# Autodesk Inventor assembly: Wheel 42T and 34T
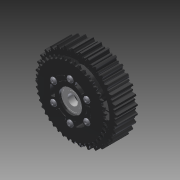
[picture p0: Inventor's stored thumbnail of the model, 180x180]
Saved by Autodesk Inventor 2013 (Build 170138000, 138)
## iProperties
Created: 2013-02-02
Part Number: Wheel 42T and 34T
Document SubType Name: Assembly
Designer: Niemitalo_Dan
Author: Niemitalo_Dan
## Documents named in this file (7)
- \\lmss\STUDENTS\Robotics\CAD Files\COTS Parts\Kit Frame - VexPro\Wheel 42T and 34T drive in a day.iam
- \\lmss\STUDENTS\Robotics\CAD Files\COTS Parts\Wheels\VexPro VersaWheel 4in.ipt
- \\lmss\STUDENTS\Robotics\CAD Files\COTS Parts\Sprockets - VexPro #25\25 Sprocket 34T Vex.ipt
- \\lmss\STUDENTS\Robotics\CAD Files\COTS Parts\Sprockets - VexPro #25\25 Sprocket 42T Vex.ipt
- \\lmss\STUDENTS\Robotics\CAD Files\COTS Parts\Fasteners\8-32 locknut.ipt
- \\lmss\STUDENTS\Robotics\CAD Files\COTS Parts\Fasteners\8-32 BHCS x2000.ipt
- \\lmss\STUDENTS\Robotics\CAD Files\COTS Parts\Bearings - VexPro\Flanged Bearing - 0.5in Round ID x 1.125in OD.ipt
## Components (17 placed, 6 different names)
1. VexPro VersaWheel 4in:1 — Mate:1, Mate:2, Mate:3, Mate:4, Mate:5, Mate:6, Mate:7, Mate:8, Mate:9, Mate:10
2. 25 Sprocket 34T Vex:1 — Mate:1, Mate:2, Mate:3, Insert:3
3. 25 Sprocket 42T Vex:1 — Mate:4, Mate:5, Mate:6, Insert:4
4. Flanged Bearing - 0.5in Round ID x 1.125in OD:1 — Mate:7, Mate:8
5. Flanged Bearing - 0.5in Round ID x 1.125in OD:2 — Mate:9, Mate:10
6. 8-32 BHCS x2000:1 — Insert:4
7. 8-32 locknut:1 — Insert:3
8. 8-32 BHCS x2000:2
9. 8-32 locknut:2
10. 8-32 BHCS x2000:3
11. 8-32 locknut:3
12. 8-32 BHCS x2000:4
13. 8-32 locknut:4
14. 8-32 BHCS x2000:5
15. 8-32 locknut:5
16. 8-32 BHCS x2000:6
17. 8-32 locknut:6
## Component patterns: (6 elements, first: 8-32 BHCS x2000:1 + 8-32 locknut:1)
## Relationships (12: Mate 10, Insert 2)
- Mate:1: VexPro VersaWheel 4in:1 ↔ 25 Sprocket 34T Vex:1
- Mate:2: VexPro VersaWheel 4in:1 ↔ 25 Sprocket 34T Vex:1
- Mate:3: VexPro VersaWheel 4in:1 ↔ 25 Sprocket 34T Vex:1
- Mate:4: VexPro VersaWheel 4in:1 ↔ 25 Sprocket 42T Vex:1
- Mate:5: VexPro VersaWheel 4in:1 ↔ 25 Sprocket 42T Vex:1
- Mate:6: VexPro VersaWheel 4in:1 ↔ 25 Sprocket 42T Vex:1
- Insert:3: 25 Sprocket 34T Vex:1 ↔ 8-32 locknut:1
- Insert:4: 25 Sprocket 42T Vex:1 ↔ 8-32 BHCS x2000:1
- Mate:7: VexPro VersaWheel 4in:1 ↔ Flanged Bearing - 0.5in Round ID x 1.125in OD:1
- Mate:8: VexPro VersaWheel 4in:1 ↔ Flanged Bearing - 0.5in Round ID x 1.125in OD:1
- Mate:9: VexPro VersaWheel 4in:1 ↔ Flanged Bearing - 0.5in Round ID x 1.125in OD:2
- Mate:10: VexPro VersaWheel 4in:1 ↔ Flanged Bearing - 0.5in Round ID x 1.125in OD:2
